# Autodesk Inventor assembly: right
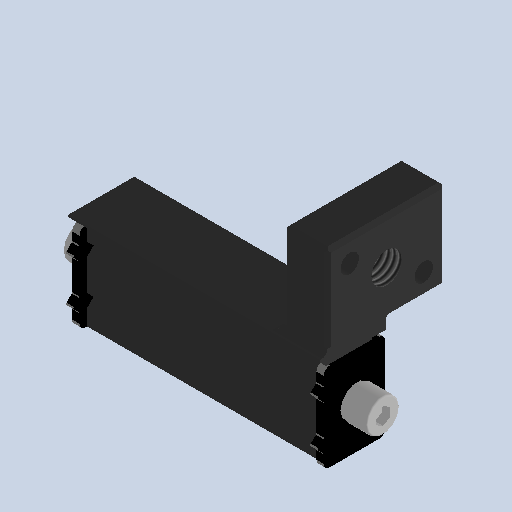
[picture p0: Inventor's stored thumbnail of the model, 512x512]
Saved by Autodesk Inventor 2023 (Build 270158000, 158)
## iProperties
Created: 2022-09-14
Part Number: right
Document SubType Name: Assembly
Designer: Robert
Author: Robert
## Documents named in this file (4)
- C:\Users\Rober\Documents\Ingenieurinformatik\grop\catkin\src\grop\coactegpc\urdf\40\base\ktoe\right.iam
- C:\Users\Rober\Documents\Ingenieurinformatik\grop\catkin\src\grop\coactegpc\urdf\40\base\ktoe\SCHUNK-5521119 Finger EGP 40.ipt
- C:\Users\Rober\Documents\Ingenieurinformatik\grop\catkin\src\grop\coactegpc\urdf\40\base\ktoe\SCHUNK-9962713 Bracket MPG 40.ipt
- C:\Users\Rober\Documents\Ingenieurinformatik\grop\catkin\src\grop\coactegpc\urdf\40\base\ktoe\SCHUNK-9965221-Scheibe D4_5.ipt
## Components (5 placed, 3 different names)
1. SCHUNK-5521119 Finger EGP 40:1
2. SCHUNK-9962713 Bracket MPG 40:1
3. SCHUNK-9965221-Scheibe D4_5:1
4. SCHUNK-9962713 Bracket MPG 40:2
5. SCHUNK-9965221-Scheibe D4_5:2
## Relationships (12: Mate 5, Angle 4, Flush 3)
- [Flush]: SCHUNK-5521119 Finger EGP 40:1 ↔ SCHUNK-9962713 Bracket MPG 40:1
- [Mate]: SCHUNK-5521119 Finger EGP 40:1 ↔ SCHUNK-9962713 Bracket MPG 40:1
- [Angle] (0 deg): SCHUNK-5521119 Finger EGP 40:1 ↔ SCHUNK-9962713 Bracket MPG 40:1
- [Flush]: SCHUNK-9962713 Bracket MPG 40:1 ↔ SCHUNK-9965221-Scheibe D4_5:1
- [Mate]: SCHUNK-9962713 Bracket MPG 40:1 ↔ SCHUNK-9965221-Scheibe D4_5:1
- [Angle] (0 deg): SCHUNK-9962713 Bracket MPG 40:1 ↔ SCHUNK-9965221-Scheibe D4_5:1
- [Mate]: SCHUNK-5521119 Finger EGP 40:1 ↔ SCHUNK-9962713 Bracket MPG 40:2
- [Mate]: SCHUNK-5521119 Finger EGP 40:1 ↔ SCHUNK-9962713 Bracket MPG 40:2
- [Angle] (0 deg): SCHUNK-5521119 Finger EGP 40:1 ↔ SCHUNK-9962713 Bracket MPG 40:2
- [Flush]: SCHUNK-9962713 Bracket MPG 40:2 ↔ SCHUNK-9965221-Scheibe D4_5:2
- [Mate]: SCHUNK-9962713 Bracket MPG 40:2 ↔ SCHUNK-9965221-Scheibe D4_5:2
- [Angle] (0 deg): SCHUNK-9962713 Bracket MPG 40:2 ↔ SCHUNK-9965221-Scheibe D4_5:2
